# Autodesk Inventor assembly: DOBLE PUENTE H
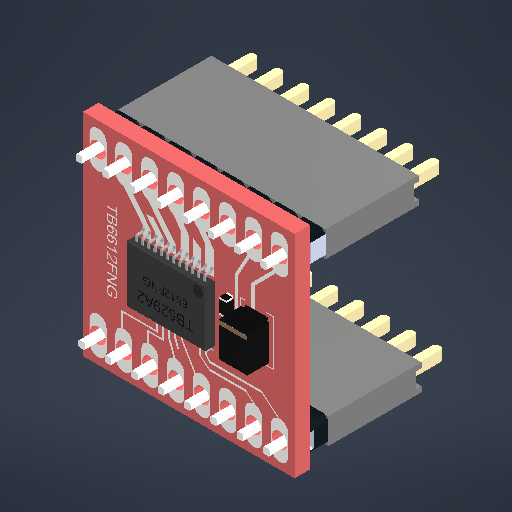
[picture p0: Inventor's stored thumbnail of the model, 512x512]
Saved by Autodesk Inventor 2026.1 (Build 301233020, 233B)
## iProperties
Created: 2019-11-22
Part Number: DOBLE PUENTE H
Document SubType Name: Assembly
Designer: celio
Sending System: Autodesk Translation Framework v8.12.0.6
Preprocessor: ST-DEVELOPER v18
Title: C:/Users/CDMX Electrónica/Desktop/DOBLE PUENTE H.step
## Documents named in this file (7)
- C:\Users\celio\OneDrive\Documentos\Inventor\ZeGuia\Componentes\Ponte H\TB6612FNG\TB6612FNG.iam
- C:\Users\celio\OneDrive\Documentos\Inventor\ZeGuia\Componentes\Ponte H\TB6612FNG\parts\TB6612FNG v6.ipt
- C:\Users\celio\OneDrive\Documentos\Inventor\ZeGuia\Componentes\Ponte H\TB6612FNG\parts\capacitor v2.ipt
- C:\Users\celio\OneDrive\Documentos\Inventor\ZeGuia\Componentes\Ponte H\TB6612FNG\parts\capacitor_v1 v5.ipt
- C:\Users\celio\OneDrive\Documentos\Inventor\ZeGuia\Componentes\Ponte H\TB6612FNG\parts\header_8 v1.ipt
- C:\Users\celio\OneDrive\Documentos\Inventor\ZeGuia\Componentes\Ponte H\TB6612FNG\parts\Peça42.ipt
- C:\Users\celio\OneDrive\Documentos\Inventor\ZeGuia\Pinos\Femea\1x8\1x8.ipt
## Components (9 placed, 6 different names)
1. TB6612FNG v6:1
2. capacitor v2:1
3. capacitor_v1 v5:1
4. capacitor_v1 v5:2
5. header_8 v1:1 — Coincidente:2, Alinhado:3, Alinhado:4
6. header_8 v1:2 — Coincidente:1, Alinhado:1, Alinhado:2
7. Peça42
8. 1x8:1 — Coincidente:1, Alinhado:1, Alinhado:2
9. 1x8:2 — Coincidente:2, Alinhado:3, Alinhado:4
## Relationships (6: Flush 4, Mate 2)
- Coincidente:1 [Mate]: header_8 v1:2 ↔ 1x8:1
- Alinhado:1 [Flush]: header_8 v1:2 ↔ 1x8:1
- Alinhado:2 [Flush]: header_8 v1:2 ↔ 1x8:1
- Coincidente:2 [Mate]: header_8 v1:1 ↔ 1x8:2
- Alinhado:3 [Flush]: header_8 v1:1 ↔ 1x8:2
- Alinhado:4 [Flush]: header_8 v1:1 ↔ 1x8:2
